# Autodesk Inventor assembly: EndStop
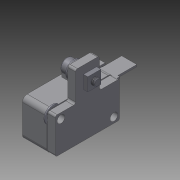
[picture p0: Inventor's stored thumbnail of the model, 180x180]
Saved by Autodesk Inventor 2014 (Build 180170000, 170)
## iProperties
Created: 2014-10-17
Part Number: EndStop
Document SubType Name: Assembly
Designer: ThatOtherGuy
Author: ThatOtherGuy
## Documents named in this file (6)
- C:\Users\ThatOtherGuy\Documents\Inventor\KosselCNC1515\Frame\EndStop.iam
- C:\Users\ThatOtherGuy\Documents\Inventor\KosselCNC1515\Frame\EndStop_Bracket.ipt
- C:\Users\ThatOtherGuy\Documents\Inventor\KosselCNC1515\Frame\EndStop_LimitSwitch.ipt
- C:\Users\ThatOtherGuy\Documents\Inventor\Content Center Files\R2014\en-US\DIN 125-1  A\DIN 125 - A 3.2.ipt
- C:\Users\ThatOtherGuy\Documents\Inventor\Content Center Files\R2014\en-US\DIN 562\DIN 562 - M3 x 5.5.ipt
- C:\Users\ThatOtherGuy\Documents\Inventor\Content Center Files\R2014\en-US\ANSI B18.3.1M(1)\ANSI B18.3.1M - M3x0.5 x 12(2).ipt
## Components (5 placed, 5 different names)
1. EndStop_Bracket:1 — Mate:1, Mate:2, Mate:3, Insert:1, Mate:5, Angle:1, Mate:6
2. EndStop_LimitSwitch:1 — Mate:1, Mate:2, Mate:3
3. DIN 125-1 A A 3.2:1 — Insert:1, Mate:7
4. Broached Socket Head Cap Screw - Metric M3x0.5 x 12:1 — Mate:4, Mate:6, Mate:7
5. DIN 562 M3:1 — Mate:4, Mate:5, Angle:1
## Relationships (9: Mate 7, Insert 1, Angle 1)
- Mate:1: EndStop_Bracket:1 ↔ EndStop_LimitSwitch:1
- Mate:2: EndStop_Bracket:1 ↔ EndStop_LimitSwitch:1
- Mate:3: EndStop_Bracket:1 ↔ EndStop_LimitSwitch:1
- Insert:1: EndStop_Bracket:1 ↔ DIN 125-1 A A 3.2:1
- Mate:4: Broached Socket Head Cap Screw - Metric M3x0.5 x 12:1 ↔ DIN 562 M3:1
- Mate:5 (1.1 mm): EndStop_Bracket:1 ↔ DIN 562 M3:1
- Angle:1 (0 deg): EndStop_Bracket:1 ↔ DIN 562 M3:1
- Mate:6: EndStop_Bracket:1 ↔ Broached Socket Head Cap Screw - Metric M3x0.5 x 12:1
- Mate:7: DIN 125-1 A A 3.2:1 ↔ Broached Socket Head Cap Screw - Metric M3x0.5 x 12:1
